# Autodesk Inventor assembly: wally
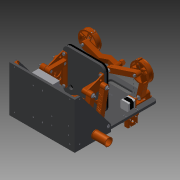
[picture p0: Inventor's stored thumbnail of the model, 180x180]
Saved by Autodesk Inventor 2014 (Build 180170000, 170)
## iProperties
Created: 2013-10-14
Part Number: wally
Document SubType Name: Assembly
Designer: employee
Author: employee
## Documents named in this file (25)
- \\GRISTLE\speco\GitHub\ConceptFORGE\Wally\wally.iam
- \\GRISTLE\speco\GitHub\ConceptFORGE\Wally\back board.ipt
- \\GRISTLE\speco\GitHub\ConceptFORGE\Wally\z arm wall bracket.iam
- \\GRISTLE\speco\GitHub\ConceptFORGE\Wally\xy mount.iam
- \\GRISTLE\speco\GitHub\ConceptFORGE\Wally\corner tab.iam
- \\GRISTLE\speco\GitHub\ConceptFORGE\Wally\bottom.ipt
- \\GRISTLE\speco\GitHub\ConceptFORGE\Wally\side support1.ipt
- \\GRISTLE\speco\GitHub\ConceptFORGE\Wally\side support.ipt
- \\GRISTLE\speco\GitHub\ConceptFORGE\Wally\edge tab.iam
- \\GRISTLE\speco\GitHub\ConceptFORGE\Wally\arm.iam
- \\GRISTLE\speco\GitHub\ConceptFORGE\Wally\bed bracket right.iam
- \\GRISTLE\speco\GitHub\ConceptFORGE\Wally\bed bracket right_MIR.iam
- \\GRISTLE\speco\GitHub\ConceptFORGE\Wally\bed.iam
- \\GRISTLE\speco\GitHub\ConceptFORGE\Wally\M8x70.ipt
- \\GRISTLE\speco\GitHub\ConceptFORGE\Wally\spool holder.iam
- \\GRISTLE\speco\GitHub\ConceptFORGE\Wally\M8x100.ipt
- \\GRISTLE\speco\GitHub\ConceptFORGE\Wally\standoff.iam
- \\GRISTLE\speco\GitHub\ConceptFORGE\Wally\big pulley.iam
- \\GRISTLE\speco\GitHub\ConceptFORGE\Wally\xy forearm.iam
- \\GRISTLE\speco\GitHub\ConceptFORGE\Wally\xy ubis mount arm.iam
- \\GRISTLE\speco\GitHub\ConceptFORGE\Wally\ubis.ipt
- \\GRISTLE\speco\GitHub\ConceptFORGE\Wally\z motor.iam
- \\GRISTLE\speco\GitHub\ConceptFORGE\Wally\power supply.iam
- \\GRISTLE\speco\GitHub\ConceptFORGE\Wally\filament drive.iam
- \\GRISTLE\speco\GitHub\ConceptFORGE\Wally\small pulley.iam
## Components (37 placed, 24 different names)
1. back board:1 — Mate:1, Mate:2, Flush:1, Insert:1, Insert:2, Insert:3, Insert:4, Insert:5, Insert:6, Insert:7, Insert:8, Insert:9, Angle:1, Insert:10, Angle:2, Insert:44, Mate:6, Insert:48, Mate:8
2. z arm wall bracket:1 [sub-assembly] — Insert:1, Insert:2, Mate:4, Insert:23, Insert:24
3. z arm wall bracket:2 [sub-assembly] — Insert:3, Insert:4, Mate:3, Insert:21, Insert:22
4. xy mount:1 [sub-assembly] — Insert:5, Insert:7, Insert:19, Insert:49
5. xy mount:2 [sub-assembly] — Insert:6, Insert:8, Insert:20, Insert:50
6. corner tab:1 [sub-assembly] — Insert:9, Angle:1, Insert:11, Insert:13
7. corner tab:2 [sub-assembly] — Insert:10, Angle:2, Insert:12, Insert:14
8. bottom:1 — Insert:11, Insert:12, Insert:17, Insert:18, Insert:45, Insert:46, Insert:47, Mate:7
9. side support1:1 — Insert:14, Mate:3, Insert:16, Insert:33, Insert:34, Angle:3
10. side support:1 — Insert:13, Mate:4, Insert:15, Insert:31, Insert:32
11. edge tab:1 [sub-assembly] — Insert:16, Insert:18
12. edge tab:2 [sub-assembly] — Insert:15, Insert:17
13. arm:1 [sub-assembly] — Insert:21, Insert:25
14. arm:2 [sub-assembly] — Insert:24, Insert:27
15. arm:3 [sub-assembly] — Insert:23, Insert:28
16. arm:4 [sub-assembly] — Insert:22, Insert:26
17. arm:5 [sub-assembly] — Insert:19, Insert:37
18. arm:6 [sub-assembly] — Insert:20, Insert:38
19. bed bracket right:1 [sub-assembly] — Insert:25, Insert:26, Insert:30
20. bed bracket right_MIR:1 [sub-assembly] — Insert:27, Insert:28, Insert:29
21. bed:1 [sub-assembly] — Insert:29, Insert:30
22. Hex Bolt - Metric M8 x 1.25 x 70:2 — Insert:31
23. Hex Bolt - Metric M8 x 1.25 x 70:3 — Insert:32
24. Hex Bolt - Metric M8 x 1.25 x 70:4 — Insert:33
25. spool holder:1 [sub-assembly] — Insert:34, Insert:35
26. M8x100 — Insert:35, Angle:3
27. standoff:1 [sub-assembly] — Insert:45, Insert:46
28. big pulley:1 [sub-assembly] — Insert:37, Insert:39, Insert:40, Mate:10
29. big pulley:2 [sub-assembly] — Insert:38, Insert:41, Insert:42, Mate:9
30. xy forearm:1 [sub-assembly] — Insert:39, Insert:40, Mate:5
31. xy ubis mount arm:1 [sub-assembly] — Insert:41, Mate:5, Insert:42, Insert:43
32. ubis:1 — Insert:43
33. z motor:1 [sub-assembly] — Insert:44, Mate:6
34. power supply:1 [sub-assembly] — Insert:47, Mate:7
35. filament drive:1 [sub-assembly] — Insert:48, Mate:8
36. small pulley:1 [sub-assembly] — Insert:49, Mate:10
37. small pulley:2 [sub-assembly] — Insert:50, Mate:9
## Relationships (63: Insert 49, Mate 10, Angle 3, Flush 1)
- Mate:1: back board:1
- Mate:2: back board:1
- Flush:1: back board:1
- Insert:1: back board:1 ↔ z arm wall bracket:1
- Insert:2: back board:1 ↔ z arm wall bracket:1
- Insert:3: back board:1 ↔ z arm wall bracket:2
- Insert:4: back board:1 ↔ z arm wall bracket:2
- Insert:5: back board:1 ↔ xy mount:1
- Insert:6: back board:1 ↔ xy mount:2
- Insert:7: back board:1 ↔ xy mount:1
- Insert:8: back board:1 ↔ xy mount:2
- Insert:9: back board:1 ↔ corner tab:1
- Angle:1 (0 deg): back board:1 ↔ corner tab:1
- Insert:10: back board:1 ↔ corner tab:2
- Angle:2 (0 deg): back board:1 ↔ corner tab:2
- Insert:11: corner tab:1 ↔ bottom:1
- Insert:12: corner tab:2 ↔ bottom:1
- Insert:13: corner tab:1 ↔ side support:1
- Insert:14: corner tab:2 ↔ side support1:1
- Mate:3: z arm wall bracket:2 ↔ side support1:1
- Mate:4: z arm wall bracket:1 ↔ side support:1
- Insert:15: side support:1 ↔ edge tab:2
- Insert:16: side support1:1 ↔ edge tab:1
- Insert:17: bottom:1 ↔ edge tab:2
- Insert:18: bottom:1 ↔ edge tab:1
- Insert:19: xy mount:1 ↔ arm:5
- Insert:20: xy mount:2 ↔ arm:6
- Insert:21: z arm wall bracket:2 ↔ arm:1
- Insert:22: z arm wall bracket:2 ↔ arm:4
- Insert:23: z arm wall bracket:1 ↔ arm:3
- Insert:24: z arm wall bracket:1 ↔ arm:2
- Insert:25: arm:1 ↔ bed bracket right:1
- Insert:26: arm:4 ↔ bed bracket right:1
- Insert:27: arm:2 ↔ bed bracket right_MIR:1
- Insert:28: arm:3 ↔ bed bracket right_MIR:1
- Insert:29: bed bracket right_MIR:1 ↔ bed:1
- Insert:30: bed bracket right:1 ↔ bed:1
- Insert:31: side support:1 ↔ Hex Bolt - Metric M8 x 1.25 x 70:2
- Insert:32: side support:1 ↔ Hex Bolt - Metric M8 x 1.25 x 70:3
- Insert:33: side support1:1 ↔ Hex Bolt - Metric M8 x 1.25 x 70:4
- Insert:34: side support1:1 ↔ spool holder:1
- Insert:35: spool holder:1 ↔ M8x100
- Angle:3 (0 deg): side support1:1 ↔ M8x100
- Insert:37: arm:5 ↔ big pulley:1
- Insert:38: arm:6 ↔ big pulley:2
- Insert:39: big pulley:1 ↔ xy forearm:1
- Insert:40: big pulley:1 ↔ xy forearm:1
- Insert:41: big pulley:2 ↔ xy ubis mount arm:1
- Mate:5: xy forearm:1 ↔ xy ubis mount arm:1
- Insert:42: big pulley:2 ↔ xy ubis mount arm:1
- Insert:43: xy ubis mount arm:1 ↔ ubis:1
- Insert:44: back board:1 ↔ z motor:1
- Mate:6: back board:1 ↔ z motor:1
- Insert:45: bottom:1 ↔ standoff:1
- Insert:46: bottom:1 ↔ standoff:1
- Insert:47: bottom:1 ↔ power supply:1
- Mate:7: bottom:1 ↔ power supply:1
- Insert:48: back board:1 ↔ filament drive:1
- Mate:8: back board:1 ↔ filament drive:1
- Insert:49: xy mount:1 ↔ small pulley:1
- Insert:50: xy mount:2 ↔ small pulley:2
- Mate:9: big pulley:2 ↔ small pulley:2
- Mate:10: big pulley:1 ↔ small pulley:1
